# Autodesk Inventor assembly: Assembly
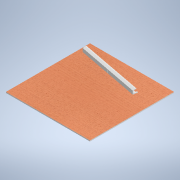
[picture p0: Inventor's stored thumbnail of the model, 180x180]
Saved by Autodesk Inventor 2020 (Build 240168000, 168)
## iProperties
Created: 2020-02-20
Part Number: Assembly
Document SubType Name: Assembly
Designer: brand
Author: brand
## Documents named in this file (3)
- C:\Users\brand\Documents\Longhorn 3D Printing\Week1\Assembly.iam
- C:\Users\brand\Documents\Longhorn 3D Printing\Week1\Base.ipt
- C:\Users\brand\Documents\Longhorn 3D Printing\Week1\StraightTrackv2_v0.ipt
## Components (3 placed, 2 different names)
1. Base:1 — Mate:1, Mate:2
2. StraightTrackv2_v0:1 — Mate:1, Mate:3, Flush:1
3. StraightTrackv2_v0:2 — Mate:2, Mate:3, Flush:1
## Relationships (4: Mate 3, Flush 1)
- Mate:1: Base:1 ↔ StraightTrackv2_v0:1
- Mate:2: Base:1 ↔ StraightTrackv2_v0:2
- Mate:3: StraightTrackv2_v0:1 ↔ StraightTrackv2_v0:2
- Flush:1: StraightTrackv2_v0:1 ↔ StraightTrackv2_v0:2
